# Autodesk Inventor assembly: Holder
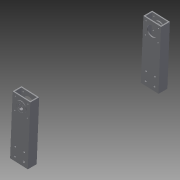
[picture p0: Inventor's stored thumbnail of the model, 180x180]
Saved by Autodesk Inventor 2013 (Build 170138000, 138)
## iProperties
Created: 2014-01-24
Part Number: Holder
Document SubType Name: Assembly
Designer: Jarod
Author: Jarod
## Documents named in this file (3)
- E:\Robotics\FRC\2014\CAD\Robot\Pickup\Z-Holder.iam
- E:\Robotics\FRC\2014\CAD\Robot\Pickup\Z-Bar.ipt
- E:\Robotics\FRC\2014\CAD\Robot\Pickup\BigBearing.ipt
## Components (4 placed, 2 different names)
1. Z-Bar:1 — Flush:1, Flush:2, Mate:1, Mate:8, Mate:10
2. Z-Bar:2 — Flush:1, Flush:2, Mate:1, Mate:9, Mate:11
3. BigBearing:1 — Mate:8, Mate:10
4. BigBearing:2 — Mate:9, Mate:11
## Relationships (7: Mate 5, Flush 2)
- Flush:1: Z-Bar:1 ↔ Z-Bar:2
- Flush:2: Z-Bar:1 ↔ Z-Bar:2
- Mate:1 (349.25 mm): Z-Bar:1 ↔ Z-Bar:2
- Mate:8: Z-Bar:1 ↔ BigBearing:1
- Mate:9: Z-Bar:2 ↔ BigBearing:2
- Mate:10: Z-Bar:1 ↔ BigBearing:1
- Mate:11: Z-Bar:2 ↔ BigBearing:2
